# Autodesk Inventor assembly: AssemblyGripper
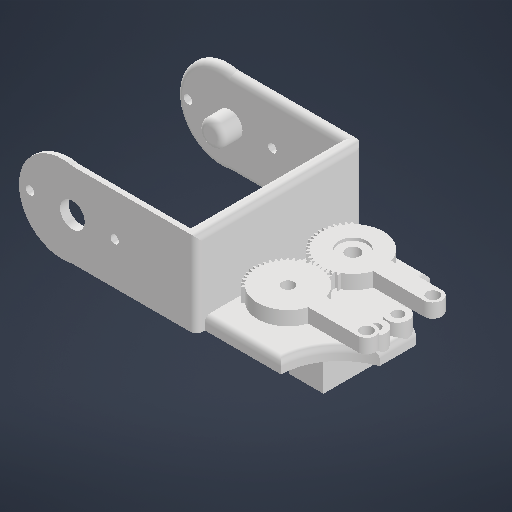
[picture p0: Inventor's stored thumbnail of the model, 512x512]
Saved by Autodesk Inventor 2026.2 (Build 302298000, 298)
## iProperties
Created: 2026-04-07
Part Number: AssemblyGripper
Document SubType Name: Assembly
Designer: Brian Wang
Author: Brian Wang
## Documents named in this file (5)
- C:\Users\Brian Wang\Downloads\RoboticsChess\3D_Model\gripper\AssemblyGripper.iam
- C:\Users\Brian Wang\Downloads\RoboticsChess\3D_Model\gripper\innerGearL.ipt
- C:\Users\Brian Wang\Downloads\RoboticsChess\3D_Model\gripper\innerGearR.ipt
- C:\Users\Brian Wang\Downloads\RoboticsChess\3D_Model\gripper\main.ipt
- C:\Users\Brian Wang\Downloads\RoboticsChess\3D_Model\gripper\testingservo.ipt
## Components (4 placed, 4 different names)
1. main:1 — Mate:1, Mate:2, Mate:3, Cylindrical:1
2. testingservo:1 — Mate:1, Mate:2, Mate:3, Cylindrical:2
3. innerGearL:1 — Cylindrical:1
4. innerGearR:1 — Cylindrical:2
## Relationships (5: Mate 3, CylindricalJoint 2)
- Mate:1: main:1 ↔ testingservo:1
- Mate:2: main:1 ↔ testingservo:1
- Mate:3: main:1 ↔ testingservo:1
- Cylindrical:1: main:1 ↔ innerGearL:1
- Cylindrical:2: testingservo:1 ↔ innerGearR:1
